# Autodesk Inventor assembly: espejos de la mot
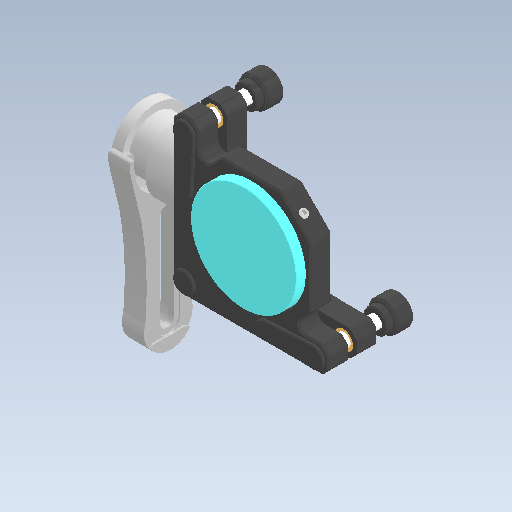
[picture p0: Inventor's stored thumbnail of the model, 512x512]
Saved by Autodesk Inventor 2020 (Build 240168000, 168)
## iProperties
Created: 2022-10-18
Part Number: espejos de la mot
Document SubType Name: Assembly
Designer: General
Author: General
## Documents named in this file (4)
- C:\LAFriOC\diseños\sistema de vacío\Ensambles\espejos de la mot.iam
- C:\LAFriOC\diseños\sistema de vacío\KM200-E03-Solidworks.ipt
- C:\LAFriOC\diseños\sistema de vacío\Óptica para la MOT\Espejo inferior y base\POSTE_ESPEJO.ipt
- C:\LAFriOC\diseños\sistema de vacío\CF175-Solidworks.ipt
## Components (3 placed, 3 different names)
1. KM200-E03-Solidworks:1 — Insertar:1
2. POSTE_ESPEJO:1 — Insertar:1, Insertar:2
3. CF175-Solidworks:1 — Insertar:2
## Relationships (2: Insert 2)
- Insertar:1: KM200-E03-Solidworks:1 ↔ POSTE_ESPEJO:1
- Insertar:2: POSTE_ESPEJO:1 ↔ CF175-Solidworks:1
